# Autodesk Inventor assembly: robot
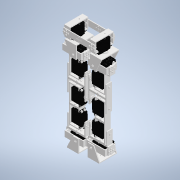
[picture p0: Inventor's stored thumbnail of the model, 180x180]
Saved by Autodesk Inventor 2021.4 (Build 254397000, 397)
## iProperties
Created: 2022-07-24
Part Number: robot
Document SubType Name: Assembly
Designer: isamu
Author: isamu
## Documents named in this file (12)
- D:\personal_projects\robot\inventor\2021_matlab_compat\robot.iam
- D:\personal_projects\robot\inventor\2021_matlab_compat\mg996r_two_servo_bottom_middle.iam
- D:\personal_projects\robot\inventor\2021_matlab_compat\mg996r_left_mid_top_two_servo.iam
- D:\personal_projects\robot\inventor\2021_matlab_compat\mg996r_rot_into_rot.iam
- D:\personal_projects\robot\inventor\2021_matlab_compat\mg996r_left_rot_foot_servo.iam
- D:\personal_projects\robot\inventor\2021_matlab_compat\mg996r_left_foot_frame.iam
- D:\personal_projects\robot\inventor\2021_matlab_compat\mg996r_right_rot_foot_servo.iam
- D:\personal_projects\robot\inventor\2021_matlab_compat\mg996r_right_foot_frame.iam
- D:\personal_projects\robot\inventor\2021_matlab_compat\mg996r_right_mid_top_two_servo.iam
- D:\personal_projects\robot\inventor\2021_matlab_compat\mg996r_right_top_rot_frame.iam
- D:\personal_projects\robot\inventor\2021_matlab_compat\mg996r_left_top_rot_frame.iam
- D:\personal_projects\robot\inventor\2021_matlab_compat\mg996r_top_two_servo_v1.iam
## Components (13 placed, 11 different names)
1. mg996r_left_mid_top_two_servo:1 [sub-assembly] — Mate:1, Mate:2, Mate:17, Mate:18
2. mg996r_rot_into_rot:1 [sub-assembly] — Mate:1, Mate:2, Mate:3, Mate:4
3. mg996r_two_servo_bottom_middle:1 [sub-assembly] — Mate:3, Mate:4, Mate:5, Mate:6
4. mg996r_left_rot_foot_servo:1 [sub-assembly] — Mate:5, Mate:6, Mate:7, Mate:8
5. mg996r_left_foot_frame:1 [sub-assembly] — Mate:7, Mate:8
6. mg996r_two_servo_bottom_middle:2 [sub-assembly] — Mate:9, Mate:10, Mate:11, Mate:12
7. mg996r_rot_into_rot:2 [sub-assembly] — Mate:9, Mate:10, Mate:15, Mate:16
8. mg996r_right_rot_foot_servo:1 [sub-assembly] — Mate:11, Mate:12, Mate:13, Mate:14
9. mg996r_right_foot_frame:1 [sub-assembly] — Mate:13, Mate:14
10. mg996r_right_mid_top_two_servo:1 [sub-assembly] — Mate:15, Mate:16, Mate:21, Mate:22
11. mg996r_right_top_rot_frame:1 [sub-assembly] — Mate:21, Mate:22, Mate:23, Mate:24
12. mg996r_left_top_rot_frame:2 [sub-assembly] — Mate:17, Mate:18, Mate:19, Mate:20
13. mg996r_top_two_servo_v1:1 [sub-assembly] — Mate:19, Mate:20, Mate:23, Mate:24
## Relationships (24: Mate 24)
- Mate:1: mg996r_left_mid_top_two_servo:1 ↔ mg996r_rot_into_rot:1
- Mate:2: mg996r_left_mid_top_two_servo:1 ↔ mg996r_rot_into_rot:1
- Mate:3: mg996r_rot_into_rot:1 ↔ mg996r_two_servo_bottom_middle:1
- Mate:4: mg996r_rot_into_rot:1 ↔ mg996r_two_servo_bottom_middle:1
- Mate:5: mg996r_two_servo_bottom_middle:1 ↔ mg996r_left_rot_foot_servo:1
- Mate:6: mg996r_two_servo_bottom_middle:1 ↔ mg996r_left_rot_foot_servo:1
- Mate:7: mg996r_left_rot_foot_servo:1 ↔ mg996r_left_foot_frame:1
- Mate:8: mg996r_left_rot_foot_servo:1 ↔ mg996r_left_foot_frame:1
- Mate:9: mg996r_two_servo_bottom_middle:2 ↔ mg996r_rot_into_rot:2
- Mate:10: mg996r_two_servo_bottom_middle:2 ↔ mg996r_rot_into_rot:2
- Mate:11: mg996r_two_servo_bottom_middle:2 ↔ mg996r_right_rot_foot_servo:1
- Mate:12: mg996r_two_servo_bottom_middle:2 ↔ mg996r_right_rot_foot_servo:1
- Mate:13: mg996r_right_rot_foot_servo:1 ↔ mg996r_right_foot_frame:1
- Mate:14: mg996r_right_rot_foot_servo:1 ↔ mg996r_right_foot_frame:1
- Mate:15: mg996r_rot_into_rot:2 ↔ mg996r_right_mid_top_two_servo:1
- Mate:16: mg996r_rot_into_rot:2 ↔ mg996r_right_mid_top_two_servo:1
- Mate:17: mg996r_left_mid_top_two_servo:1 ↔ mg996r_left_top_rot_frame:2
- Mate:18: mg996r_left_mid_top_two_servo:1 ↔ mg996r_left_top_rot_frame:2
- Mate:19: mg996r_left_top_rot_frame:2 ↔ mg996r_top_two_servo_v1:1
- Mate:20: mg996r_left_top_rot_frame:2 ↔ mg996r_top_two_servo_v1:1
- Mate:21: mg996r_right_mid_top_two_servo:1 ↔ mg996r_right_top_rot_frame:1
- Mate:22: mg996r_right_mid_top_two_servo:1 ↔ mg996r_right_top_rot_frame:1
- Mate:23: mg996r_right_top_rot_frame:1 ↔ mg996r_top_two_servo_v1:1
- Mate:24: mg996r_right_top_rot_frame:1 ↔ mg996r_top_two_servo_v1:1
